# Autodesk Inventor assembly: main
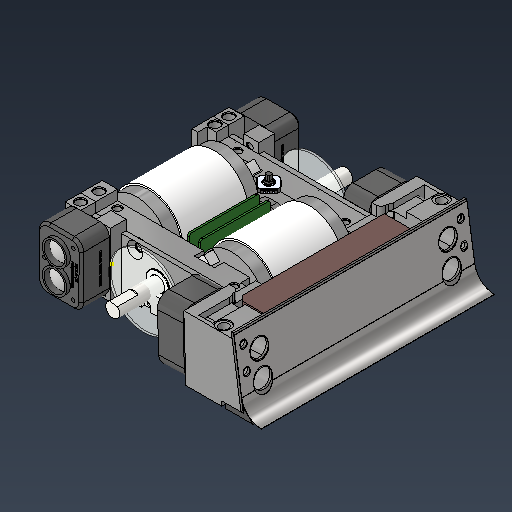
[picture p0: Inventor's stored thumbnail of the model, 512x512]
Saved by Autodesk Inventor 2026.2 (Build 302298010, 298A)
## iProperties
Created: 2026-03-09
Part Number: main
Document SubType Name: Assembly
Designer: szymo
Mass: 408.789 g
Surface Area: 1162.1 cm^2
Volume: 160.791 cm^3
Density: 2.54237 g/cm^3
Author: szymo
## Documents named in this file (21)
- D:\tech\robotyka\robots\evangelion-turbo\inventor-project\main.iam
- D:\tech\robotyka\robots\evangelion-turbo\inventor-project\drive-train.iam
- D:\tech\robotyka\robots\evangelion-turbo\inventor-project\LUNA.ipt
- D:\tech\robotyka\robots\evangelion-turbo\inventor-project\3s450mah.ipt
- D:\tech\robotyka\robots\evangelion-turbo\inventor-project\KTIR-Board.ipt
- D:\tech\robotyka\robots\evangelion-turbo\inventor-project\plug.ipt
- D:\tech\robotyka\robots\evangelion-turbo\inventor-project\FonrtMount.ipt
- D:\tech\robotyka\robots\evangelion-turbo\inventor-project\0.96 oled\0.96 oled\0.96 oled.ipt
- D:\tech\robotyka\robots\evangelion-turbo\inventor-project\THMU 13 (SMD JOYSTICK)\THMU 13 (SMD JOYSTICK)\THMU 13 (SMD JOYSTICK).ipt
- D:\tech\robotyka\robots\evangelion-turbo\inventor-project\SteelFront.ipt
- D:\tech\robotyka\robots\evangelion-turbo\inventor-project\SpringSteelFront.ipt
- D:\tech\robotyka\robots\evangelion-turbo\inventor-project\LeftGearbox.ipt
- D:\tech\robotyka\robots\evangelion-turbo\inventor-project\LeftGearboxCoverr.ipt
- D:\tech\robotyka\robots\evangelion-turbo\inventor-project\RightGearbox.ipt
- D:\tech\robotyka\robots\evangelion-turbo\inventor-project\RightGearboxCover.ipt
- D:\tech\robotyka\robots\evangelion-turbo\inventor-project\GearboxBearingHolderCover.ipt
- D:\tech\robotyka\robots\evangelion-turbo\inventor-project\PCBs_Holder.ipt
- D:\tech\robotyka\robots\evangelion-turbo\inventor-project\GearboxBearingHolderCover_MIR.ipt
- D:\tech\robotyka\robots\evangelion-turbo\inventor-project\PCB_Main.ipt
- D:\tech\robotyka\robots\evangelion-turbo\inventor-project\PCB_InterfaceBoard.ipt
- D:\tech\robotyka\robots\evangelion-turbo\inventor-project\1703 Fan asm\1703 Fan asm\1703 Fan asm.ipt
## Components (27 placed, 20 different names)
1. drive-train:1 [sub-assembly] — Flush:2, Flush:3, Flush:4, Mate:2, Mate:3, Tangent:1, Mate:18, Mate:23
2. 3s450mah:1 — Flush:8, Tangent:1, Flush:9
3. LUNA:2 — Mate:1, Mate:3, Angle:2, Mate:11
4. LUNA:1 — Flush:5, Mate:2, Angle:1, Mate:12
5. LUNA:3 — Flush:22, Flush:23, Mate:6
6. LUNA:4 — Flush:24, Flush:25, Mate:7
7. KTIR-Board:1 — Flush:10, Flush:11, Flush:13
8. KTIR-Board:2 — Mate:4, Flush:12, Flush:14
9. KTIR-Board:4 — Flush:17, Flush:27, Mate:6, Mate:18
10. KTIR-Board:5 — Flush:28, Flush:29, Mate:7, Mate:19
11. SpringSteelFront:1 — Flush:65, Mate:21, Mate:22
12. SteelFront:1 — Flush:62
13. plug:1 — Mate:10, Flush:45, Mate:20
14. FonrtMount:1 — Flush:47
15. GearboxBearingHolderCover:1 — Flush:74
16. LeftGearbox:1 — Flush:67
17. LeftGearboxCoverr:1 — Flush:69
18. RightGearboxCover:1 — Flush:73
19. RightGearbox:1 — Flush:71, Flush:80
20. GearboxBearingHolderCover_MIR:1 — Mate:23, Flush:78, Flush:79
21. 1703 Fan asm:1 — Mate:30, Mate:31, Mate:32
22. PCB_Main:1 — Mate:24, Mate:25, Mate:29
23. PCB_Main:2 — Mate:26, Mate:27, Mate:28
24. PCBs_Holder:1 — Flush:77, Mate:24, Mate:25, Mate:26, Mate:27, Mate:28, Mate:29, Mate:30, Mate:31, Mate:32
25. PCB_InterfaceBoard:1 — Flush:80
26. THMU 13 (SMD JOYSTICK):1
27. 0.96 oled:1
## Relationships (64: Flush 37, Mate 24, Angle 2, Tangent 1)
- Flush:2: drive-train:1
- Flush:3 (-19.2 mm): drive-train:1
- Flush:4: drive-train:1
- Flush:5 (49.5 mm): LUNA:1
- Mate:1 (-49.5 mm): LUNA:2
- Mate:2 (19 mm): drive-train:1 ↔ LUNA:1
- Mate:3 (19 mm): drive-train:1 ↔ LUNA:2
- Angle:1 (-2 deg): LUNA:1
- Angle:2 (182 deg): LUNA:2
- Flush:8 (4.5 mm): 3s450mah:1
- Tangent:1: drive-train:1 ↔ 3s450mah:1
- Flush:9 (-31.5 mm): 3s450mah:1
- Flush:10 (-46.5 mm): KTIR-Board:1
- Mate:4 (-46.5 mm): KTIR-Board:2
- Flush:11 (0.13 mm): KTIR-Board:1
- Flush:12 (0.13 mm): KTIR-Board:2
- Flush:13 (66.673 mm): KTIR-Board:1
- Flush:14 (-66.673 mm): KTIR-Board:2
- Flush:17: KTIR-Board:4
- Flush:22: LUNA:3
- Flush:23 (1 mm): LUNA:3
- Flush:24 (1 mm): LUNA:4
- Flush:25: LUNA:4
- Flush:27 (1 mm): KTIR-Board:4
- Flush:28 (1 mm): KTIR-Board:5
- Flush:29: KTIR-Board:5
- Mate:6: LUNA:3 ↔ KTIR-Board:4
- Mate:7: LUNA:4 ↔ KTIR-Board:5
- Mate:10: plug:1
- Flush:45: plug:1
- Mate:11: LUNA:2
- Mate:12: LUNA:1
- Flush:47: FonrtMount:1
- Flush:53 (-29 mm)
- Mate:18: drive-train:1 ↔ KTIR-Board:4
- Mate:19 (19.2 mm): KTIR-Board:5
- Flush:62: SteelFront:1
- Mate:20 (-95.5 mm): plug:1
- Flush:65: SpringSteelFront:1
- Mate:21: SpringSteelFront:1
- Mate:22: SpringSteelFront:1
- Flush:66 (-19.2 mm)
- Flush:67: LeftGearbox:1
- Flush:68 (-28.5 mm)
- Flush:69: LeftGearboxCoverr:1
- Flush:70 (19.2 mm)
- Flush:71: RightGearbox:1
- Flush:72 (28.5 mm)
- Flush:73: RightGearboxCover:1
- Flush:74: GearboxBearingHolderCover:1
- Flush:77: PCBs_Holder:1
- Mate:23: drive-train:1 ↔ GearboxBearingHolderCover_MIR:1
- Flush:78: GearboxBearingHolderCover_MIR:1
- Flush:79 (3 mm): GearboxBearingHolderCover_MIR:1
- Mate:24: PCB_Main:1 ↔ PCBs_Holder:1
- Mate:25: PCB_Main:1 ↔ PCBs_Holder:1
- Mate:26: PCB_Main:2 ↔ PCBs_Holder:1
- Mate:27: PCB_Main:2 ↔ PCBs_Holder:1
- Mate:28: PCB_Main:2 ↔ PCBs_Holder:1
- Mate:29: PCB_Main:1 ↔ PCBs_Holder:1
- Flush:80: RightGearbox:1 ↔ PCB_InterfaceBoard:1
- Mate:30: 1703 Fan asm:1 ↔ PCBs_Holder:1
- Mate:31 (0.25 mm): 1703 Fan asm:1 ↔ PCBs_Holder:1
- Mate:32 (0.25 mm): 1703 Fan asm:1 ↔ PCBs_Holder:1
